# Autodesk Inventor assembly: joint3_as
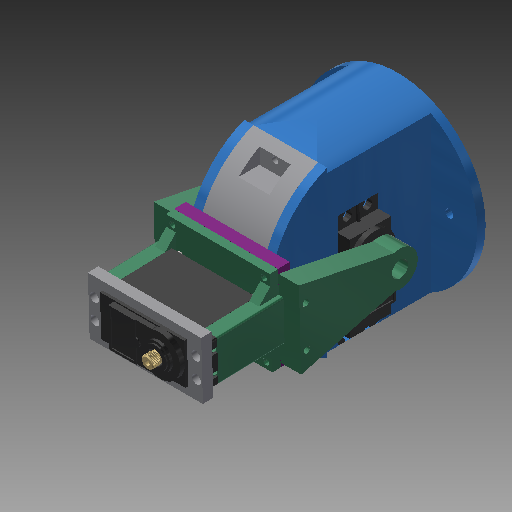
[picture p0: Inventor's stored thumbnail of the model, 512x512]
Saved by Autodesk Inventor 2019 (Build 230136000, 136)
## iProperties
Created: 2019-12-29
Part Number: joint3_as
Material: Типовые
Document SubType Name: Assembly
Designer: Петров Иван
Author: Петров Иван
## Documents named in this file (7)
- E:\IVAN\Ivan_desktop\GitHub\Arm_manip\hardware\МД.001.800 - Звено 3.iam
- E:\IVAN\Ivan_desktop\GitHub\Arm_manip\hardware\МД.001.801 - Основа.ipt
- E:\IVAN\Ivan_desktop\GitHub\Arm_manip\hardware\Standart_things\tower prone.ipt
- E:\IVAN\Ivan_desktop\GitHub\Arm_manip\hardware\МД.001.802 - Рычаг.ipt
- E:\IVAN\Ivan_desktop\GitHub\Arm_manip\hardware\МД.001.803 - Скользящая пластина.ipt
- E:\IVAN\Ivan_desktop\GitHub\Arm_manip\hardware\МД.001.804 - Крышка.ipt
- E:\IVAN\Ivan_desktop\GitHub\Arm_manip\hardware\МД.001.1000 - Захват.iam
## Components (7 placed, 6 different names)
1. МД.001.801 - Основа:1 — Совмещение:1, Совмещение:2, Совмещение:3, Совмещение:6, Совмещение:7, Совмещение:12, Совмещение:13, Совмещение:14
2. tower prone:1 — Совмещение:1, Совмещение:2, Совмещение:3, Совмещение:4, Совмещение:5
3. МД.001.802 - Рычаг:1 — Совмещение:4, Совмещение:5, Совмещение:9, Заподлицо:1, Совмещение:15, Совмещение:16
4. МД.001.802 - Рычаг:2 — Совмещение:6, Совмещение:7, Совмещение:17, Совмещение:18
5. МД.001.803 - Скользящая пластина:1 — Совмещение:9, Заподлицо:1, Совмещение:15, Совмещение:16, Совмещение:17, Совмещение:18, Совмещение:19, Совмещение:20, Совмещение:21
6. МД.001.804 - Крышка:1 — Совмещение:12, Совмещение:13, Совмещение:14
7. МД.001.1000 - Захват:1 [sub-assembly] — Совмещение:19, Совмещение:20, Совмещение:21
## Relationships (19: Mate 18, Flush 1)
- Совмещение:1 [Mate]: МД.001.801 - Основа:1 ↔ tower prone:1
- Совмещение:2 [Mate]: МД.001.801 - Основа:1 ↔ tower prone:1
- Совмещение:3 [Mate]: МД.001.801 - Основа:1 ↔ tower prone:1
- Совмещение:4 [Mate]: tower prone:1 ↔ МД.001.802 - Рычаг:1
- Совмещение:5 [Mate]: tower prone:1 ↔ МД.001.802 - Рычаг:1
- Совмещение:6 [Mate]: МД.001.801 - Основа:1 ↔ МД.001.802 - Рычаг:2
- Совмещение:7 [Mate]: МД.001.801 - Основа:1 ↔ МД.001.802 - Рычаг:2
- Совмещение:9 [Mate]: МД.001.802 - Рычаг:1 ↔ МД.001.803 - Скользящая пластина:1
- Заподлицо:1 [Flush]: МД.001.802 - Рычаг:1 ↔ МД.001.803 - Скользящая пластина:1
- Совмещение:12 [Mate]: МД.001.801 - Основа:1 ↔ МД.001.804 - Крышка:1
- Совмещение:13 [Mate]: МД.001.801 - Основа:1 ↔ МД.001.804 - Крышка:1
- Совмещение:14 [Mate]: МД.001.801 - Основа:1 ↔ МД.001.804 - Крышка:1
- Совмещение:15 [Mate]: МД.001.802 - Рычаг:1 ↔ МД.001.803 - Скользящая пластина:1
- Совмещение:16 [Mate]: МД.001.802 - Рычаг:1 ↔ МД.001.803 - Скользящая пластина:1
- Совмещение:17 [Mate]: МД.001.802 - Рычаг:2 ↔ МД.001.803 - Скользящая пластина:1
- Совмещение:18 [Mate]: МД.001.802 - Рычаг:2 ↔ МД.001.803 - Скользящая пластина:1
- Совмещение:19 [Mate]: МД.001.803 - Скользящая пластина:1 ↔ МД.001.1000 - Захват:1
- Совмещение:20 [Mate]: МД.001.803 - Скользящая пластина:1 ↔ МД.001.1000 - Захват:1
- Совмещение:21 [Mate]: МД.001.803 - Скользящая пластина:1 ↔ МД.001.1000 - Захват:1
